# Autodesk Inventor assembly: Link_02_Assembly
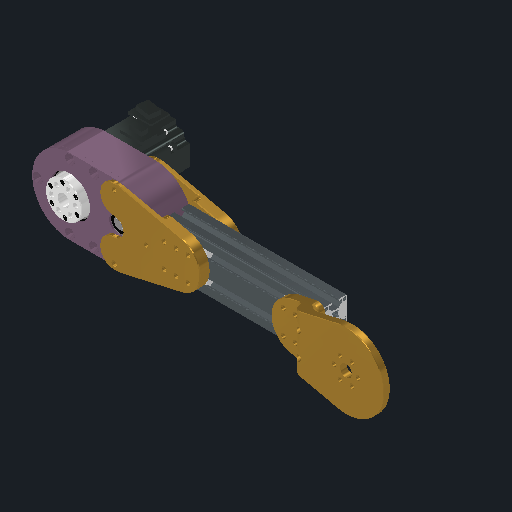
[picture p0: Inventor's stored thumbnail of the model, 512x512]
Saved by Autodesk Inventor 2026 (Build 300175000, 175)
## iProperties
Created: 2025-11-30
Part Number: Link_02_Assembly
Document SubType Name: Assembly
Designer: pochi
Mass: 1919.36 g
Surface Area: 3767.02 cm^2
Volume: 936.563 cm^3
Density: 2.04936 g/cm^3
Author: pochi
## Documents named in this file (5)
- D:\POLIMI\3RD SEMESTER\Industrial Robotics\Project\Mine\Link_02_Assembly.iam
- D:\POLIMI\3RD SEMESTER\Industrial Robotics\Project\Mine\Link_02.ipt
- D:\POLIMI\3RD SEMESTER\Industrial Robotics\Project\Mine\RotationalConector_30x60.ipt
- D:\POLIMI\3RD SEMESTER\Industrial Robotics\Project\Mine\RigidConector_30x60.ipt
- D:\POLIMI\3RD SEMESTER\Industrial Robotics\Project\Mine\Reducer.iam
## Components (5 placed, 4 different names)
1. Link_02:1 — Mate:1, Mate:2, Mate:3, Mate:4, Mate:5, Mate:6, Mate:7, Mate:8, Mate:9
2. RotationalConector_30x60:1 — Mate:1, Mate:2, Mate:3
3. RigidConector_30x60:1 — Mate:4, Mate:5, Mate:6, Mate:11, Mate:12
4. RigidConector_30x60:2 — Mate:7, Mate:8, Mate:9, Mate:10
5. Reducer:1 [sub-assembly] — Mate:10, Mate:11, Mate:12
## Relationships (12: Mate 12)
- Mate:1: Link_02:1 ↔ RotationalConector_30x60:1
- Mate:2: Link_02:1 ↔ RotationalConector_30x60:1
- Mate:3: Link_02:1 ↔ RotationalConector_30x60:1
- Mate:4: Link_02:1 ↔ RigidConector_30x60:1
- Mate:5: Link_02:1 ↔ RigidConector_30x60:1
- Mate:6: Link_02:1 ↔ RigidConector_30x60:1
- Mate:7: Link_02:1 ↔ RigidConector_30x60:2
- Mate:8: Link_02:1 ↔ RigidConector_30x60:2
- Mate:9: Link_02:1 ↔ RigidConector_30x60:2
- Mate:10: RigidConector_30x60:2 ↔ Reducer:1
- Mate:11: RigidConector_30x60:1 ↔ Reducer:1
- Mate:12: RigidConector_30x60:1 ↔ Reducer:1
